# Autodesk Inventor assembly: Intake Full Assembly
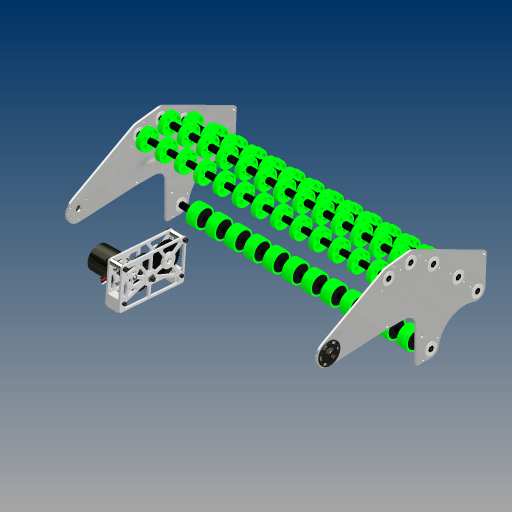
[picture p0: Inventor's stored thumbnail of the model, 512x512]
Saved by Autodesk Inventor 2024.3 (Build 283343000, 343)
## iProperties
Created: 2024-07-29
Part Number: Intake Full Assembly
Document SubType Name: Assembly
Designer: Kenji
Author: Kenji
## Documents named in this file (8)
- C:\Users\Kenji\Documents\GitHub\1622-2024-Summer-CAD-A-Thon\Intake\Intake Full Assembly.iam
- C:\Users\Kenji\Documents\GitHub\1622-2024-Summer-CAD-A-Thon\Intake\Intake Roller Plate.ipt
- C:\Users\Kenji\Documents\GitHub\1622-2024-Summer-CAD-A-Thon\COTS Library\Motion\Bearings\COTS_WCP-0783_1.125ODHexBearing.ipt
- C:\Users\Kenji\Documents\GitHub\1622-2024-Summer-CAD-A-Thon\Intake\Intake HexShaft 1.ipt
- C:\Users\Kenji\Documents\GitHub\1622-2024-Summer-CAD-A-Thon\COTS Library\Motion\Wheels\Compliant Wheels\2in compliant wheels\0.500in hex bore\COTS_am-3462_2indiameter_0.500inhexbore_durometer35A_CompliantWheel.ipt
- C:\Users\Kenji\Documents\GitHub\1622-2024-Summer-CAD-A-Thon\COTS Library\Motion\Wheels\Stealth Wheels\COTS_am-3155 2IN 500Hex Stealth Wheel.iam
- C:\Users\Kenji\Documents\GitHub\1622-2024-Summer-CAD-A-Thon\Intake\Intake Pivot Assembly.iam
- C:\Users\Kenji\Documents\GitHub\1622-2024-Summer-CAD-A-Thon\COTS Library\Structural Adapter\VersaHubs\COTS_217-2592_VersaHub.ipt
## Components (100 placed, 7 different names)
1. Intake Roller Plate:1 — Mate:111, Mate:112, Mate:113, Mate:114, Mate:116, Mate:117, Mate:119, Mate:120, Mate:121, Mate:122, Mate:123, Mate:124, Mate:125, Mate:137, Mate:138, Mate:139, Mate:140
2. Intake Roller Plate:2 — Mate:116, Mate:117, Mate:118, Mate:126, Mate:127, Mate:128, Mate:129, Mate:141, Mate:142, Mate:143, Mate:145
3. COTS_WCP-0783_1.125ODHexBearing:1 — Mate:25, Mate:32, Flush:11, Mate:128, Mate:129
4. COTS_WCP-0783_1.125ODHexBearing:2 — Mate:26, Mate:27, Flush:1
5. COTS_WCP-0783_1.125ODHexBearing:3 — Mate:31, Flush:9
6. COTS_WCP-0783_1.125ODHexBearing:4 — Flush:8, Mate:126, Mate:127
7. COTS_WCP-0783_1.125ODHexBearing:5 — Flush:4, Mate:118
8. COTS_WCP-0783_1.125ODHexBearing:6 — Flush:6, Mate:145
9. COTS_WCP-0783_1.125ODHexBearing:7 — Flush:10, Mate:111, Mate:115, Mate:124, Mate:125, Mate:135
10. COTS_WCP-0783_1.125ODHexBearing:8 — Mate:30, Flush:7, Mate:122, Mate:123, Mate:130
11. COTS_WCP-0783_1.125ODHexBearing:9 — Mate:29, Flush:5, Mate:112, Mate:121, Mate:134
12. COTS_WCP-0783_1.125ODHexBearing:10 — Mate:25, Flush:12, Mate:136
13. COTS_WCP-0783_1.125ODHexBearing:11 — Mate:26, Flush:2, Mate:114, Mate:119, Mate:132, Mate:144
14. COTS_WCP-0783_1.125ODHexBearing:12 — Mate:28, Flush:3, Mate:33, Mate:113, Mate:120, Mate:133
15. Intake HexShaft 1:1 — Mate:31, Flush:9, Flush:10, Mate:85, Mate:115
16. Intake HexShaft 1:2 — Mate:32, Flush:11, Flush:12, Mate:98
17. Intake HexShaft 1:3 — Mate:30, Flush:7, Flush:8, Mate:72
18. Intake HexShaft 1:4 — Mate:29, Flush:5, Flush:6, Mate:59
19. Intake HexShaft 1:5 — Mate:28, Flush:3, Flush:4
20. Intake HexShaft 1:6 — Mate:27, Flush:1, Flush:2
21. Intake Pivot Assembly:1 [sub-assembly] — Mate:137
22. COTS_217-2592_VersaHub:2 — Mate:138, Mate:139, Mate:140
23. COTS_217-2592_VersaHub:3 — Mate:141, Mate:142, Mate:143
24. COTS_am-3462_2indiameter_0.500inhexbore_durometer35A_CompliantWheel:66 — Mate:98, Mate:136
25. COTS_am-3462_2indiameter_0.500inhexbore_durometer35A_CompliantWheel:40 — Mate:72, Mate:130
26. COTS_am-3462_2indiameter_0.500inhexbore_durometer35A_CompliantWheel:53 — Mate:85, Mate:135
27. COTS_am-3462_2indiameter_0.500inhexbore_durometer35A_CompliantWheel:25 — Mate:59, Mate:134
28. COTS_am-3462_2indiameter_0.500inhexbore_durometer35A_CompliantWheel:24 — Mate:33, Mate:133
29. COTS_am-3462_2indiameter_0.500inhexbore_durometer35A_CompliantWheel:67
30. COTS_am-3462_2indiameter_0.500inhexbore_durometer35A_CompliantWheel:68
31. COTS_am-3462_2indiameter_0.500inhexbore_durometer35A_CompliantWheel:69
32. COTS_am-3462_2indiameter_0.500inhexbore_durometer35A_CompliantWheel:70
33. COTS_am-3462_2indiameter_0.500inhexbore_durometer35A_CompliantWheel:71
34. COTS_am-3462_2indiameter_0.500inhexbore_durometer35A_CompliantWheel:72
35. COTS_am-3462_2indiameter_0.500inhexbore_durometer35A_CompliantWheel:73
36. COTS_am-3462_2indiameter_0.500inhexbore_durometer35A_CompliantWheel:74
37. COTS_am-3462_2indiameter_0.500inhexbore_durometer35A_CompliantWheel:75
38. COTS_am-3462_2indiameter_0.500inhexbore_durometer35A_CompliantWheel:76
39. COTS_am-3462_2indiameter_0.500inhexbore_durometer35A_CompliantWheel:77
40. COTS_am-3462_2indiameter_0.500inhexbore_durometer35A_CompliantWheel:78
41. COTS_am-3462_2indiameter_0.500inhexbore_durometer35A_CompliantWheel:79
42. COTS_am-3462_2indiameter_0.500inhexbore_durometer35A_CompliantWheel:80
43. COTS_am-3462_2indiameter_0.500inhexbore_durometer35A_CompliantWheel:81
44. COTS_am-3462_2indiameter_0.500inhexbore_durometer35A_CompliantWheel:82
45. COTS_am-3462_2indiameter_0.500inhexbore_durometer35A_CompliantWheel:83
46. COTS_am-3462_2indiameter_0.500inhexbore_durometer35A_CompliantWheel:84
47. COTS_am-3462_2indiameter_0.500inhexbore_durometer35A_CompliantWheel:85
48. COTS_am-3462_2indiameter_0.500inhexbore_durometer35A_CompliantWheel:86
49. COTS_am-3462_2indiameter_0.500inhexbore_durometer35A_CompliantWheel:87
50. COTS_am-3462_2indiameter_0.500inhexbore_durometer35A_CompliantWheel:88
51. COTS_am-3462_2indiameter_0.500inhexbore_durometer35A_CompliantWheel:89
52. COTS_am-3462_2indiameter_0.500inhexbore_durometer35A_CompliantWheel:90
53. COTS_am-3462_2indiameter_0.500inhexbore_durometer35A_CompliantWheel:91
54. COTS_am-3462_2indiameter_0.500inhexbore_durometer35A_CompliantWheel:92
55. COTS_am-3462_2indiameter_0.500inhexbore_durometer35A_CompliantWheel:93
56. COTS_am-3462_2indiameter_0.500inhexbore_durometer35A_CompliantWheel:94
57. COTS_am-3462_2indiameter_0.500inhexbore_durometer35A_CompliantWheel:95
58. COTS_am-3462_2indiameter_0.500inhexbore_durometer35A_CompliantWheel:96
59. COTS_am-3462_2indiameter_0.500inhexbore_durometer35A_CompliantWheel:97
60. COTS_am-3462_2indiameter_0.500inhexbore_durometer35A_CompliantWheel:98
61. COTS_am-3462_2indiameter_0.500inhexbore_durometer35A_CompliantWheel:99
62. COTS_am-3462_2indiameter_0.500inhexbore_durometer35A_CompliantWheel:100
63. COTS_am-3462_2indiameter_0.500inhexbore_durometer35A_CompliantWheel:101
64. COTS_am-3462_2indiameter_0.500inhexbore_durometer35A_CompliantWheel:102
65. COTS_am-3462_2indiameter_0.500inhexbore_durometer35A_CompliantWheel:103
66. COTS_am-3462_2indiameter_0.500inhexbore_durometer35A_CompliantWheel:104
67. COTS_am-3462_2indiameter_0.500inhexbore_durometer35A_CompliantWheel:105
68. COTS_am-3462_2indiameter_0.500inhexbore_durometer35A_CompliantWheel:106
69. COTS_am-3462_2indiameter_0.500inhexbore_durometer35A_CompliantWheel:107
70. COTS_am-3462_2indiameter_0.500inhexbore_durometer35A_CompliantWheel:108
71. COTS_am-3462_2indiameter_0.500inhexbore_durometer35A_CompliantWheel:109
72. COTS_am-3462_2indiameter_0.500inhexbore_durometer35A_CompliantWheel:110
73. COTS_am-3462_2indiameter_0.500inhexbore_durometer35A_CompliantWheel:111
74. COTS_am-3462_2indiameter_0.500inhexbore_durometer35A_CompliantWheel:112
75. COTS_am-3462_2indiameter_0.500inhexbore_durometer35A_CompliantWheel:113
76. COTS_am-3462_2indiameter_0.500inhexbore_durometer35A_CompliantWheel:114
77. COTS_am-3462_2indiameter_0.500inhexbore_durometer35A_CompliantWheel:115
78. COTS_am-3462_2indiameter_0.500inhexbore_durometer35A_CompliantWheel:116
79. COTS_am-3462_2indiameter_0.500inhexbore_durometer35A_CompliantWheel:117
80. COTS_am-3462_2indiameter_0.500inhexbore_durometer35A_CompliantWheel:118
81. COTS_am-3462_2indiameter_0.500inhexbore_durometer35A_CompliantWheel:119
82. COTS_am-3462_2indiameter_0.500inhexbore_durometer35A_CompliantWheel:120
83. COTS_am-3462_2indiameter_0.500inhexbore_durometer35A_CompliantWheel:121
84. COTS_am-3462_2indiameter_0.500inhexbore_durometer35A_CompliantWheel:122
85. COTS_am-3462_2indiameter_0.500inhexbore_durometer35A_CompliantWheel:123
86. COTS_am-3462_2indiameter_0.500inhexbore_durometer35A_CompliantWheel:124
87. COTS_am-3462_2indiameter_0.500inhexbore_durometer35A_CompliantWheel:125
88. COTS_am-3462_2indiameter_0.500inhexbore_durometer35A_CompliantWheel:126
89. COTS_am-3155 2IN 500Hex Stealth Wheel:7 [sub-assembly] — Mate:132, Mate:144
90. COTS_am-3155 2IN 500Hex Stealth Wheel:8 [sub-assembly]
91. COTS_am-3155 2IN 500Hex Stealth Wheel:9 [sub-assembly]
92. COTS_am-3155 2IN 500Hex Stealth Wheel:10 [sub-assembly]
93. COTS_am-3155 2IN 500Hex Stealth Wheel:11 [sub-assembly]
94. COTS_am-3155 2IN 500Hex Stealth Wheel:12 [sub-assembly]
95. COTS_am-3155 2IN 500Hex Stealth Wheel:13 [sub-assembly]
96. COTS_am-3155 2IN 500Hex Stealth Wheel:14 [sub-assembly]
97. COTS_am-3155 2IN 500Hex Stealth Wheel:15 [sub-assembly]
98. COTS_am-3155 2IN 500Hex Stealth Wheel:16 [sub-assembly]
99. COTS_am-3155 2IN 500Hex Stealth Wheel:17 [sub-assembly]
100. COTS_am-3155 2IN 500Hex Stealth Wheel:18 [sub-assembly]
## Component patterns: (13 elements, first: COTS_am-3462_2indiameter_0.500inhexbore_durometer35A_CompliantWheel:66 + COTS_am-3462_2indiameter_0.500inhexbore_durometer35A_CompliantWheel:40 + COTS_am-3462_2indiameter_0.500inhexbore_durometer35A_CompliantWheel:53 + COTS_am-3462_2indiameter_0.500inhexbore_durometer35A_CompliantWheel:25 + COTS_am-3462_2indiameter_0.500inhexbore_durometer35A_CompliantWheel:24), (12 elements, first: COTS_am-3155 2IN 500Hex Stealth Wheel:7)
## Relationships (59: Mate 47, Flush 12)
- Mate:25: COTS_WCP-0783_1.125ODHexBearing:1 ↔ COTS_WCP-0783_1.125ODHexBearing:10
- Mate:26: COTS_WCP-0783_1.125ODHexBearing:2 ↔ COTS_WCP-0783_1.125ODHexBearing:11
- Mate:27: COTS_WCP-0783_1.125ODHexBearing:2 ↔ Intake HexShaft 1:6
- Flush:1: COTS_WCP-0783_1.125ODHexBearing:2 ↔ Intake HexShaft 1:6
- Flush:2: COTS_WCP-0783_1.125ODHexBearing:11 ↔ Intake HexShaft 1:6
- Mate:28: COTS_WCP-0783_1.125ODHexBearing:12 ↔ Intake HexShaft 1:5
- Flush:3: COTS_WCP-0783_1.125ODHexBearing:12 ↔ Intake HexShaft 1:5
- Flush:4: COTS_WCP-0783_1.125ODHexBearing:5 ↔ Intake HexShaft 1:5
- Mate:29: COTS_WCP-0783_1.125ODHexBearing:9 ↔ Intake HexShaft 1:4
- Flush:5: COTS_WCP-0783_1.125ODHexBearing:9 ↔ Intake HexShaft 1:4
- Flush:6: COTS_WCP-0783_1.125ODHexBearing:6 ↔ Intake HexShaft 1:4
- Mate:30: COTS_WCP-0783_1.125ODHexBearing:8 ↔ Intake HexShaft 1:3
- Flush:7: COTS_WCP-0783_1.125ODHexBearing:8 ↔ Intake HexShaft 1:3
- Flush:8: COTS_WCP-0783_1.125ODHexBearing:4 ↔ Intake HexShaft 1:3
- Mate:31: COTS_WCP-0783_1.125ODHexBearing:3 ↔ Intake HexShaft 1:1
- Flush:9: COTS_WCP-0783_1.125ODHexBearing:3 ↔ Intake HexShaft 1:1
- Flush:10: COTS_WCP-0783_1.125ODHexBearing:7 ↔ Intake HexShaft 1:1
- Mate:32: COTS_WCP-0783_1.125ODHexBearing:1 ↔ Intake HexShaft 1:2
- Flush:11: COTS_WCP-0783_1.125ODHexBearing:1 ↔ Intake HexShaft 1:2
- Flush:12: COTS_WCP-0783_1.125ODHexBearing:10 ↔ Intake HexShaft 1:2
- Mate:33: COTS_WCP-0783_1.125ODHexBearing:12 ↔ COTS_am-3462_2indiameter_0.500inhexbore_durometer35A_CompliantWheel:24
- Mate:59: Intake HexShaft 1:4 ↔ COTS_am-3462_2indiameter_0.500inhexbore_durometer35A_CompliantWheel:25
- Mate:72: Intake HexShaft 1:3 ↔ COTS_am-3462_2indiameter_0.500inhexbore_durometer35A_CompliantWheel:40
- Mate:85: Intake HexShaft 1:1 ↔ COTS_am-3462_2indiameter_0.500inhexbore_durometer35A_CompliantWheel:53
- Mate:98: Intake HexShaft 1:2 ↔ COTS_am-3462_2indiameter_0.500inhexbore_durometer35A_CompliantWheel:66
- Mate:111: Intake Roller Plate:1 ↔ COTS_WCP-0783_1.125ODHexBearing:7
- Mate:112: Intake Roller Plate:1 ↔ COTS_WCP-0783_1.125ODHexBearing:9
- Mate:113: Intake Roller Plate:1 ↔ COTS_WCP-0783_1.125ODHexBearing:12
- Mate:114: Intake Roller Plate:1 ↔ COTS_WCP-0783_1.125ODHexBearing:11
- Mate:115: COTS_WCP-0783_1.125ODHexBearing:7 ↔ Intake HexShaft 1:1
- Mate:116: Intake Roller Plate:1 ↔ Intake Roller Plate:2
- Mate:117: Intake Roller Plate:1 ↔ Intake Roller Plate:2
- Mate:118: Intake Roller Plate:2 ↔ COTS_WCP-0783_1.125ODHexBearing:5
- Mate:119: Intake Roller Plate:1 ↔ COTS_WCP-0783_1.125ODHexBearing:11
- Mate:120: Intake Roller Plate:1 ↔ COTS_WCP-0783_1.125ODHexBearing:12
- Mate:121: Intake Roller Plate:1 ↔ COTS_WCP-0783_1.125ODHexBearing:9
- Mate:122: Intake Roller Plate:1 ↔ COTS_WCP-0783_1.125ODHexBearing:8
- Mate:123: Intake Roller Plate:1 ↔ COTS_WCP-0783_1.125ODHexBearing:8
- Mate:124: Intake Roller Plate:1 ↔ COTS_WCP-0783_1.125ODHexBearing:7
- Mate:125: Intake Roller Plate:1 ↔ COTS_WCP-0783_1.125ODHexBearing:7
- Mate:126: Intake Roller Plate:2 ↔ COTS_WCP-0783_1.125ODHexBearing:4
- Mate:127: Intake Roller Plate:2 ↔ COTS_WCP-0783_1.125ODHexBearing:4
- Mate:128: Intake Roller Plate:2 ↔ COTS_WCP-0783_1.125ODHexBearing:1
- Mate:129: Intake Roller Plate:2 ↔ COTS_WCP-0783_1.125ODHexBearing:1
- Mate:130 (15.24 mm): COTS_WCP-0783_1.125ODHexBearing:8 ↔ COTS_am-3462_2indiameter_0.500inhexbore_durometer35A_CompliantWheel:40
- Mate:132 (33.02 mm): COTS_WCP-0783_1.125ODHexBearing:11 ↔ COTS_am-3155 2IN 500Hex Stealth Wheel:7
- Mate:133 (15.24 mm): COTS_WCP-0783_1.125ODHexBearing:12 ↔ COTS_am-3462_2indiameter_0.500inhexbore_durometer35A_CompliantWheel:24
- Mate:134 (15.24 mm): COTS_WCP-0783_1.125ODHexBearing:9 ↔ COTS_am-3462_2indiameter_0.500inhexbore_durometer35A_CompliantWheel:25
- Mate:135 (15.24 mm): COTS_WCP-0783_1.125ODHexBearing:7 ↔ COTS_am-3462_2indiameter_0.500inhexbore_durometer35A_CompliantWheel:53
- Mate:136 (15.24 mm): COTS_WCP-0783_1.125ODHexBearing:10 ↔ COTS_am-3462_2indiameter_0.500inhexbore_durometer35A_CompliantWheel:66
- Mate:137: Intake Roller Plate:1 ↔ Intake Pivot Assembly:1
- Mate:138: Intake Roller Plate:1 ↔ COTS_217-2592_VersaHub:2
- Mate:139: Intake Roller Plate:1 ↔ COTS_217-2592_VersaHub:2
- Mate:140: Intake Roller Plate:1 ↔ COTS_217-2592_VersaHub:2
- Mate:141: Intake Roller Plate:2 ↔ COTS_217-2592_VersaHub:3
- Mate:142: Intake Roller Plate:2 ↔ COTS_217-2592_VersaHub:3
- Mate:143: Intake Roller Plate:2 ↔ COTS_217-2592_VersaHub:3
- Mate:144: COTS_WCP-0783_1.125ODHexBearing:11 ↔ COTS_am-3155 2IN 500Hex Stealth Wheel:7
- Mate:145: Intake Roller Plate:2 ↔ COTS_WCP-0783_1.125ODHexBearing:6
